# Autodesk Inventor assembly: print-in-place
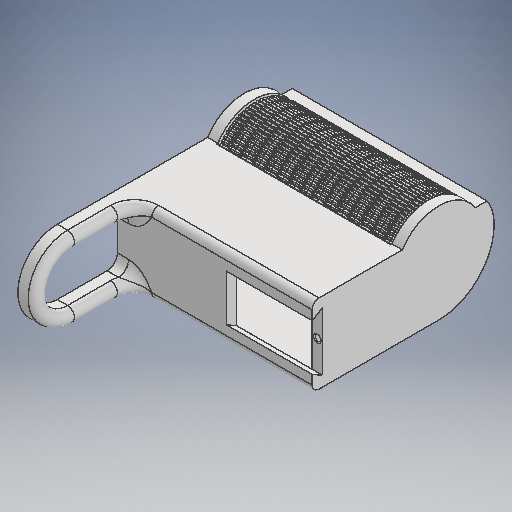
[picture p0: Inventor's stored thumbnail of the model, 512x512]
Saved by Autodesk Inventor 2025.2 (Build 292293000, 293)
## iProperties
Created: 2025-03-09
Part Number: print-in-place
Document SubType Name: Assembly
Designer: Alex
Author: Alex
## Documents named in this file (3)
- C:\Shared\alex-bartella-schoolwork\4b03\a1\a1.2\print-in-place.iam
- C:\Shared\alex-bartella-schoolwork\4b03\a1\a1.2\body.ipt
- C:\Shared\alex-bartella-schoolwork\4b03\a1\a1.2\roller.ipt
## Components (2 placed, 2 different names)
1. body:1 — Mate:1, Mate:2, Mate:3, Mate:4
2. roller:1 — Mate:2, Mate:3, Mate:4
## Relationships (4: Mate 4)
- Mate:1: body:1
- Mate:2: body:1 ↔ roller:1
- Mate:3 (0.3 mm): body:1 ↔ roller:1
- Mate:4: body:1 ↔ roller:1
